# Autodesk Inventor assembly: Assembly146-01
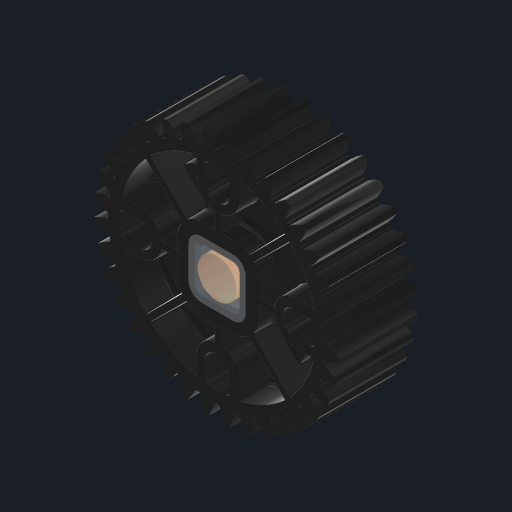
[picture p0: Inventor's stored thumbnail of the model, 512x512]
Saved by Autodesk Inventor 2024.2 (Build 282272000, 272)
## iProperties
Created: 2022-08-02
Part Number: Assembly146-01
Document SubType Name: Assembly
Designer: ylu12
Author: ylu12
## Documents named in this file (3)
- O:\cad\61002g-cad\VEX parts\Motion\Gears\HS Gear\HS 36T Gear, No Insert.iam
- O:\cad\61002g-cad\VEX parts\Motion\Gears\Reference Files\HS 36T Gear, No Insert.ipt
- O:\cad\61002g-cad\VEX parts\Motion\Gears\HS Gear.iam
## Components (1 placed, 1 different names)
1. 36T — Flush:5, Mate:9, Mate:10
## Relationships (3: Mate 2, Flush 1)
- Flush:5: 36T
- Mate:9: 36T
- Mate:10: 36T
